# Autodesk Inventor assembly: MechanumWheelLeftSubAssembly
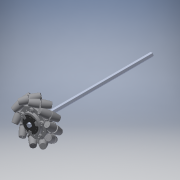
[picture p0: Inventor's stored thumbnail of the model, 180x180]
Saved by Autodesk Inventor 2017 (Build 210142000, 142)
## iProperties
Created: 2017-09-16
Part Number: MechanumWheelLeftSubAssembly
Document SubType Name: Assembly
Designer: User
Author: User
## Documents named in this file (5)
- C:\Robotics\CAD\2017-18_CAD\MechanumWheelLeftSubAssembly.iam
- C:\Robotics\CAD\COTSParts\Vex\VersaHub.5inchBore217-4009-STEP-20140807\VersaHub.5inchBore217-4009-STEP-20140807.ipt
- C:\Robotics\CAD\COTSParts\Vex\HexSprocket.5inchBore\HexSprocket18t.5inchBore217-3488-STEP\HexSprocket18t.5inchBore217-3488-STEP.ipt
- C:\Robotics\CAD\COTSParts\Vex\6inchMecanumLeft217-2799-STEP\6inchMecanumLeft217-2799.20121203.ipt
- C:\Robotics\CAD\COTSParts\Vex\HexAxle.5inchOD217-3309-STEP\HexAxle.5inchOD18inchLength217-3309-STEP.ipt
## Components (5 placed, 4 different names)
1. VersaHub.5inchBore217-4009-STEP-20140807:1 — Mate:1, Mate:2, Mate:3, Mate:7, Flush:1
2. VersaHub.5inchBore217-4009-STEP-20140807:2 — Mate:4, Mate:5, Mate:6, Mate:8
3. HexSprocket18t.5inchBore217-3488-STEP:1 — Mate:8, Mate:9, Mate:10
4. 6inchMecanumLeft217-2799.20121203:1 — Mate:1, Mate:2, Mate:3, Mate:4, Mate:5, Mate:6
5. HexAxle.5inchOD18inchLength217-3309-STEP:1 — Mate:7, Flush:1, Mate:9, Mate:10
## Relationships (11: Mate 10, Flush 1)
- Mate:1: VersaHub.5inchBore217-4009-STEP-20140807:1 ↔ 6inchMecanumLeft217-2799.20121203:1
- Mate:2: VersaHub.5inchBore217-4009-STEP-20140807:1 ↔ 6inchMecanumLeft217-2799.20121203:1
- Mate:3: VersaHub.5inchBore217-4009-STEP-20140807:1 ↔ 6inchMecanumLeft217-2799.20121203:1
- Mate:4: VersaHub.5inchBore217-4009-STEP-20140807:2 ↔ 6inchMecanumLeft217-2799.20121203:1
- Mate:5: VersaHub.5inchBore217-4009-STEP-20140807:2 ↔ 6inchMecanumLeft217-2799.20121203:1
- Mate:6: VersaHub.5inchBore217-4009-STEP-20140807:2 ↔ 6inchMecanumLeft217-2799.20121203:1
- Mate:7: VersaHub.5inchBore217-4009-STEP-20140807:1 ↔ HexAxle.5inchOD18inchLength217-3309-STEP:1
- Flush:1 (-6.35 mm): VersaHub.5inchBore217-4009-STEP-20140807:1 ↔ HexAxle.5inchOD18inchLength217-3309-STEP:1
- Mate:8 (3.175 mm): VersaHub.5inchBore217-4009-STEP-20140807:2 ↔ HexSprocket18t.5inchBore217-3488-STEP:1
- Mate:9: HexSprocket18t.5inchBore217-3488-STEP:1 ↔ HexAxle.5inchOD18inchLength217-3309-STEP:1
- Mate:10: HexSprocket18t.5inchBore217-3488-STEP:1 ↔ HexAxle.5inchOD18inchLength217-3309-STEP:1
